# Autodesk Inventor assembly: Wheel
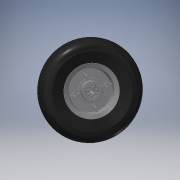
[picture p0: Inventor's stored thumbnail of the model, 180x180]
Saved by Autodesk Inventor 2018 (Build 220112000, 112)
## iProperties
Created: 2018-08-07
Part Number: Wheel
Document SubType Name: Assembly
Designer: ruben
Author: ruben
## Documents named in this file (4)
- C:\Users\ruben\Documents\Inventor\Electric-Scooter\Wheels\Wheel.iam
- C:\Users\ruben\Documents\Inventor\Electric-Scooter\!Library\76229192-9-roulement_6000_2\roulement_6000_2.iam
- C:\Users\ruben\Documents\Inventor\Electric-Scooter\Wheels\Wheel Hub.ipt
- C:\Users\ruben\Documents\Inventor\Electric-Scooter\Wheels\Wheel Tyre.ipt
## Components (4 placed, 3 different names)
1. roulement_6000_2:1 [sub-assembly] — Insert:2
2. roulement_6000_2:2 [sub-assembly] — Insert:3
3. Wheel Hub:1 — Insert:2, Insert:3, Insert:4
4. Wheel Tyre:1 — Insert:4
## Relationships (3: Insert 3)
- Insert:2: roulement_6000_2:1 ↔ Wheel Hub:1
- Insert:3: roulement_6000_2:2 ↔ Wheel Hub:1
- Insert:4: Wheel Hub:1 ↔ Wheel Tyre:1
